# Autodesk Inventor assembly: Intake
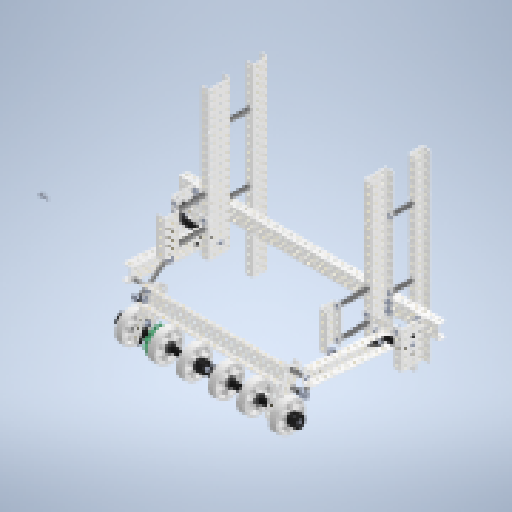
[picture p0: Inventor's stored thumbnail of the model, 512x512]
Saved by Autodesk Inventor 2023 (Build 270158000, 158)
## iProperties
Created: 2022-09-02
Part Number: Intake
Document SubType Name: Assembly
Designer: alex
Author: alex
## Documents named in this file (28)
- C:\Users\alex\Documents\GitHub\4067X_spin_up_cad\Mechanism\Intake.iam
- C:\Users\alex\Documents\GitHub\4067X_spin_up_cad\Library\Structure\Standoff\Standoff 1.00.ipt
- C:\Users\alex\Documents\GitHub\4067X_spin_up_cad\Library\Structure\Standoff.ipt
- C:\Users\alex\Documents\GitHub\4067X_spin_up_cad\Library\Structure\Standoff\Standoff 2.00.ipt
- C:\Users\alex\Documents\GitHub\4067X_spin_up_cad\Library\Structure\Hardware\Screw Steel - Star\SScrew Star Smooth .290.ipt
- C:\Users\alex\Documents\GitHub\4067X_spin_up_cad\Library\Structure\Hardware\Screw Steel - Star.ipt
- C:\Users\alex\Documents\GitHub\4067X_spin_up_cad\Library\Structure\Standoff\Standoff .50.ipt
- C:\Users\alex\Documents\GitHub\4067X_spin_up_cad\Library\Motion\Spacers\Spacer Nylon .375 OD.ipt
- C:\Users\alex\Documents\GitHub\4067X_spin_up_cad\Library\Structure\Hardware\Nut Keps.ipt
- C:\Users\alex\Documents\GitHub\4067X_spin_up_cad\Library\Motion\1-Post Bearing Flat Hex Retainer.ipt
- C:\Users\alex\Documents\GitHub\4067X_spin_up_cad\Library\Structure\Hardware\Screw Steel - Star\SScrew Star Smooth .375.ipt
- C:\Users\alex\Documents\GitHub\4067X_spin_up_cad\Library\Structure\Hardware\Nut Nylock.ipt
- C:\Users\alex\Documents\GitHub\4067X_spin_up_cad\Library\Structure\C-Channels\Aluminum 1x3x1\Alu C 1x3x1x20.ipt
- C:\Users\alex\Documents\GitHub\4067X_spin_up_cad\Library\Structure\C-Channels\Aluminum 1x3x1\Alu C 1x3x1x5.ipt
- C:\Users\alex\Documents\GitHub\4067X_spin_up_cad\Library\Structure\C-Channels\Aluminum 1x2x1\Alu C 1x2x1x35.ipt
- C:\Users\alex\Documents\GitHub\4067X_spin_up_cad\Library\Structure\Plates\Aluminum\VEX Plates\Alu Plate VEX 1x5.ipt
- C:\Users\alex\Documents\GitHub\4067X_spin_up_cad\Library\Structure\Hardware\Screw Steel - Star\SScrew Star Smooth 2.500.ipt
- C:\Users\alex\Documents\GitHub\4067X_spin_up_cad\Library\Motion\Spacers\Spacer Nylon .375 OD\NSpacer .375 OD x .375.ipt
- C:\Users\alex\Documents\GitHub\4067X_spin_up_cad\Library\Motion\Spacers\Washer Steel\SWasher .375 OD x .015625.ipt
- C:\Users\alex\Documents\GitHub\4067X_spin_up_cad\Library\Motion\Spacers\Washer Steel.ipt
- C:\Users\alex\Documents\GitHub\4067X_spin_up_cad\Library\Motion\Spacers\Spacer Nylon .375 OD\NSpacer .375 OD x .500.ipt
- C:\Users\alex\Documents\GitHub\4067X_spin_up_cad\Library\Structure\C-Channels\Aluminum 1x2x1\Alu C 1x2x1x25.ipt
- C:\Users\alex\Documents\GitHub\4067X_spin_up_cad\Library\Motion\Shaft HS\HS Bearing Flat.ipt
- C:\Users\alex\Documents\GitHub\4067X_spin_up_cad\Library\Structure\Hardware\Screw Steel - Star\SScrew Star Smooth .500.ipt
- C:\Users\alex\Documents\GitHub\4067X_spin_up_cad\Library\Structure\Hardware\Nut Thin Nylock.ipt
- C:\Users\alex\Documents\GitHub\4067X_spin_up_cad\Library\Structure\Hardware\Screw Steel - Star\SScrew Star Smooth .750.ipt
- C:\Users\alex\Documents\GitHub\4067X_spin_up_cad\Library\Structure\C-Channels\Aluminum 1x2x1\Alu C 1x2x1x5.ipt
- C:\Users\alex\Documents\GitHub\4067X_spin_up_cad\Mechanism\FloatingIntake.iam
## Components (84 placed, 23 different names)
1. Alu C 1x3x1x20:1 — Insert:105, Insert:106, Insert:109, Insert:113, Insert:115, Insert:116, Insert:117, Insert:231, Insert:234, Insert:235, Insert:238, Insert:241
2. Alu C 1x3x1x5:1 — Insert:107, Insert:108, Insert:114, Insert:120, Mate:15, Insert:145, Insert:230, Insert:244, Insert:245
3. Alu C 1x2x1x35:1 — Insert:105, Insert:106, Insert:107, Insert:108, Insert:126, Insert:127, Insert:150, Insert:151, Insert:218, Insert:219, Insert:222, Insert:223, Insert:232, Insert:233, Insert:236, Insert:237
4. Standoff 1.00:16 — Insert:109, Insert:110
5. Standoff .50:17 — Insert:110, Insert:125
6. Standoff 1.00:18 — Insert:113
7. Standoff .50:19 — Insert:124
8. Alu Plate VEX 1x5:1 — Insert:114, Insert:115, Insert:228, Insert:229
9. SScrew Star Smooth 2.500:31 — Insert:116
10. Nut Keps:3 — Insert:117, Insert:118
11. NSpacer .375 OD x .375:3 — Insert:119
12. SWasher .375 OD x .015625:1 — Insert:118, Insert:119
13. 1-Post Bearing Flat Hex Retainer:2 — Insert:120, Mate:15, Insert:146
14. NSpacer .375 OD x .500:4 — Insert:122
15. NSpacer .375 OD x .500:5 — Insert:122, Insert:123
16. NSpacer .375 OD x .375:6 — Insert:123
17. Alu C 1x2x1x25:1 — Insert:124, Insert:125, Insert:239, Insert:240
18. Alu C 1x3x1x20:2 — Insert:126, Insert:127, Insert:129, Insert:131, Insert:134, Insert:137, Insert:153, Insert:216, Insert:224, Insert:225, Insert:226, Insert:242, Insert:256, Insert:257, Mate:35
19. Standoff 1.00:20 — Insert:129
20. Standoff .50:21 — Insert:133
21. Standoff 1.00:22 — Insert:131
22. Standoff .50:23 — Insert:132
23. Alu C 1x2x1x25:2 — Insert:132, Insert:133, Insert:227, Insert:243
24. SScrew Star Smooth 2.500:32 — Insert:134, Mate:34
25. Nut Keps:4 — Insert:137
26. NSpacer .375 OD x .375:7
27. SWasher .375 OD x .015625:2
28. NSpacer .375 OD x .500:8
29. NSpacer .375 OD x .500:9
30. NSpacer .375 OD x .375:10
31. SScrew Star Smooth .375:34 — Insert:145
32. Nut Nylock:3 — Insert:146
33. Alu C 1x3x1x5:2 — Insert:150, Insert:151, Insert:152, Insert:217, Insert:220, Insert:221
34. 1-Post Bearing Flat Hex Retainer:4
35. SScrew Star Smooth .375:35
36. Nut Nylock:4
37. Alu Plate VEX 1x5:2 — Insert:152, Insert:153, Insert:214, Insert:215
38. SScrew Star Smooth .290:50 — Insert:214
39. SScrew Star Smooth .290:51 — Insert:215
40. Nut Keps:11 — Insert:216
41. Nut Keps:12 — Insert:217
42. SScrew Star Smooth .290:52 — Insert:218
43. SScrew Star Smooth .290:53 — Insert:219
44. Nut Keps:13 — Insert:220
45. Nut Keps:14 — Insert:221
46. SScrew Star Smooth .290:54 — Insert:222
47. SScrew Star Smooth .290:55 — Insert:223
48. Nut Keps:15 — Insert:224
49. Nut Keps:16 — Insert:225
50. SScrew Star Smooth .290:56 — Insert:226
51. SScrew Star Smooth .750:57 — Insert:227
52. SScrew Star Smooth .290:58 — Insert:228
53. SScrew Star Smooth .290:59 — Insert:229
54. Nut Keps:17 — Insert:230
55. Nut Keps:18 — Insert:231
56. SScrew Star Smooth .290:60 — Insert:232
57. SScrew Star Smooth .290:61 — Insert:233
58. Nut Keps:19 — Insert:234
59. Nut Keps:20 — Insert:235
60. SScrew Star Smooth .290:62 — Insert:236
61. SScrew Star Smooth .290:63 — Insert:237
62. SScrew Star Smooth .290:64 — Insert:238
63. SScrew Star Smooth .750:65 — Insert:239
64. SScrew Star Smooth .750:66 — Insert:240
65. SScrew Star Smooth .290:67 — Insert:241
66. SScrew Star Smooth .290:68 — Insert:242
67. SScrew Star Smooth .750:69 — Insert:243
68. Nut Keps:21 — Insert:244
69. Nut Keps:22 — Insert:245
70. Standoff 2.00:27 — Insert:249
71. Standoff 2.00:28 — Insert:248
72. Alu C 1x2x1x5:1 — Insert:248, Insert:249, Insert:250, Insert:251
73. SScrew Star Smooth .290:70 — Insert:250
74. SScrew Star Smooth .290:71 — Insert:251
75. Standoff 2.00:29 — Insert:256
76. Standoff 2.00:30 — Insert:257
77. Alu C 1x2x1x5:2 — Insert:259, Mate:33
78. SScrew Star Smooth .290:72
79. SScrew Star Smooth .290:73
80. HS Bearing Flat:3 — Insert:259, Mate:33, Insert:260
81. Nut Thin Nylock:3
82. SScrew Star Smooth .500:74
83. Nut Thin Nylock:4 — Insert:260
84. FloatingIntake:1 [sub-assembly] — Mate:34, Mate:35
## Relationships (94: Insert 89, Mate 5)
- Insert:105: Alu C 1x3x1x20:1 ↔ Alu C 1x2x1x35:1
- Insert:106: Alu C 1x3x1x20:1 ↔ Alu C 1x2x1x35:1
- Insert:107: Alu C 1x3x1x5:1 ↔ Alu C 1x2x1x35:1
- Insert:108: Alu C 1x3x1x5:1 ↔ Alu C 1x2x1x35:1
- Insert:109: Alu C 1x3x1x20:1 ↔ Standoff 1.00:16
- Insert:110: Standoff 1.00:16 ↔ Standoff .50:17
- [Insert]: Standoff 1.00:18 ↔ Standoff .50:19
- Insert:113: Alu C 1x3x1x20:1 ↔ Standoff 1.00:18
- Insert:114: Alu C 1x3x1x5:1 ↔ Alu Plate VEX 1x5:1
- Insert:115: Alu C 1x3x1x20:1 ↔ Alu Plate VEX 1x5:1
- Insert:116: Alu C 1x3x1x20:1 ↔ SScrew Star Smooth 2.500:31
- Insert:117: Alu C 1x3x1x20:1 ↔ Nut Keps:3
- Insert:118: Nut Keps:3 ↔ SWasher .375 OD x .015625:1
- Insert:119: NSpacer .375 OD x .375:3 ↔ SWasher .375 OD x .015625:1
- Insert:120: Alu C 1x3x1x5:1 ↔ 1-Post Bearing Flat Hex Retainer:2
- Mate:15: Alu C 1x3x1x5:1 ↔ 1-Post Bearing Flat Hex Retainer:2
- Insert:122: NSpacer .375 OD x .500:4 ↔ NSpacer .375 OD x .500:5
- Insert:123: NSpacer .375 OD x .500:5 ↔ NSpacer .375 OD x .375:6
- Insert:124: Standoff .50:19 ↔ Alu C 1x2x1x25:1
- Insert:125: Standoff .50:17 ↔ Alu C 1x2x1x25:1
- Insert:126: Alu C 1x2x1x35:1 ↔ Alu C 1x3x1x20:2
- Insert:127: Alu C 1x2x1x35:1 ↔ Alu C 1x3x1x20:2
- [Insert]: Standoff 1.00:20 ↔ Standoff .50:21
- Insert:129: Alu C 1x3x1x20:2 ↔ Standoff 1.00:20
- [Insert]: Standoff 1.00:22 ↔ Standoff .50:23
- Insert:131: Alu C 1x3x1x20:2 ↔ Standoff 1.00:22
- Insert:132: Standoff .50:23 ↔ Alu C 1x2x1x25:2
- Insert:133: Standoff .50:21 ↔ Alu C 1x2x1x25:2
- Insert:134: Alu C 1x3x1x20:2 ↔ SScrew Star Smooth 2.500:32
- [Insert]: Nut Keps:4 ↔ SWasher .375 OD x .015625:2
- [Insert]: NSpacer .375 OD x .375:7 ↔ SWasher .375 OD x .015625:2
- Insert:137: Alu C 1x3x1x20:2 ↔ Nut Keps:4
- [Insert]: NSpacer .375 OD x .500:8 ↔ NSpacer .375 OD x .500:9
- [Insert]: NSpacer .375 OD x .500:9 ↔ NSpacer .375 OD x .375:10
- Insert:145: Alu C 1x3x1x5:1 ↔ SScrew Star Smooth .375:34
- Insert:146: 1-Post Bearing Flat Hex Retainer:2 ↔ Nut Nylock:3
- [Insert]: Alu C 1x3x1x5:2 ↔ 1-Post Bearing Flat Hex Retainer:4
- [Mate]: Alu C 1x3x1x5:2 ↔ 1-Post Bearing Flat Hex Retainer:4
- [Insert]: Alu C 1x3x1x5:2 ↔ SScrew Star Smooth .375:35
- [Insert]: 1-Post Bearing Flat Hex Retainer:4 ↔ Nut Nylock:4
- Insert:150: Alu C 1x2x1x35:1 ↔ Alu C 1x3x1x5:2
- Insert:151: Alu C 1x2x1x35:1 ↔ Alu C 1x3x1x5:2
- Insert:152: Alu C 1x3x1x5:2 ↔ Alu Plate VEX 1x5:2
- Insert:153: Alu C 1x3x1x20:2 ↔ Alu Plate VEX 1x5:2
- Insert:214: Alu Plate VEX 1x5:2 ↔ SScrew Star Smooth .290:50
- Insert:215: Alu Plate VEX 1x5:2 ↔ SScrew Star Smooth .290:51
- Insert:216: Alu C 1x3x1x20:2 ↔ Nut Keps:11
- Insert:217: Alu C 1x3x1x5:2 ↔ Nut Keps:12
- Insert:218: Alu C 1x2x1x35:1 ↔ SScrew Star Smooth .290:52
- Insert:219: Alu C 1x2x1x35:1 ↔ SScrew Star Smooth .290:53
- Insert:220: Alu C 1x3x1x5:2 ↔ Nut Keps:13
- Insert:221: Alu C 1x3x1x5:2 ↔ Nut Keps:14
- Insert:222: Alu C 1x2x1x35:1 ↔ SScrew Star Smooth .290:54
- Insert:223: Alu C 1x2x1x35:1 ↔ SScrew Star Smooth .290:55
- Insert:224: Alu C 1x3x1x20:2 ↔ Nut Keps:15
- Insert:225: Alu C 1x3x1x20:2 ↔ Nut Keps:16
- Insert:226: Alu C 1x3x1x20:2 ↔ SScrew Star Smooth .290:56
- Insert:227: Alu C 1x2x1x25:2 ↔ SScrew Star Smooth .750:57
- Insert:228: Alu Plate VEX 1x5:1 ↔ SScrew Star Smooth .290:58
- Insert:229: Alu Plate VEX 1x5:1 ↔ SScrew Star Smooth .290:59
- Insert:230: Alu C 1x3x1x5:1 ↔ Nut Keps:17
- Insert:231: Alu C 1x3x1x20:1 ↔ Nut Keps:18
- Insert:232: Alu C 1x2x1x35:1 ↔ SScrew Star Smooth .290:60
- Insert:233: Alu C 1x2x1x35:1 ↔ SScrew Star Smooth .290:61
- Insert:234: Alu C 1x3x1x20:1 ↔ Nut Keps:19
- Insert:235: Alu C 1x3x1x20:1 ↔ Nut Keps:20
- Insert:236: Alu C 1x2x1x35:1 ↔ SScrew Star Smooth .290:62
- Insert:237: Alu C 1x2x1x35:1 ↔ SScrew Star Smooth .290:63
- Insert:238: Alu C 1x3x1x20:1 ↔ SScrew Star Smooth .290:64
- Insert:239: Alu C 1x2x1x25:1 ↔ SScrew Star Smooth .750:65
- Insert:240: Alu C 1x2x1x25:1 ↔ SScrew Star Smooth .750:66
- Insert:241: Alu C 1x3x1x20:1 ↔ SScrew Star Smooth .290:67
- Insert:242: Alu C 1x3x1x20:2 ↔ SScrew Star Smooth .290:68
- Insert:243: Alu C 1x2x1x25:2 ↔ SScrew Star Smooth .750:69
- Insert:244: Alu C 1x3x1x5:1 ↔ Nut Keps:21
- Insert:245: Alu C 1x3x1x5:1 ↔ Nut Keps:22
- [Insert]: Alu C 1x3x1x20:1 ↔ Standoff 2.00:27
- [Insert]: Alu C 1x3x1x20:1 ↔ Standoff 2.00:28
- Insert:248: Standoff 2.00:28 ↔ Alu C 1x2x1x5:1
- Insert:249: Standoff 2.00:27 ↔ Alu C 1x2x1x5:1
- Insert:250: Alu C 1x2x1x5:1 ↔ SScrew Star Smooth .290:70
- Insert:251: Alu C 1x2x1x5:1 ↔ SScrew Star Smooth .290:71
- [Insert]: Standoff 2.00:30 ↔ Alu C 1x2x1x5:2
- [Insert]: Standoff 2.00:29 ↔ Alu C 1x2x1x5:2
- [Insert]: Alu C 1x2x1x5:2 ↔ SScrew Star Smooth .290:72
- [Insert]: Alu C 1x2x1x5:2 ↔ SScrew Star Smooth .290:73
- Insert:256: Alu C 1x3x1x20:2 ↔ Standoff 2.00:29
- Insert:257: Alu C 1x3x1x20:2 ↔ Standoff 2.00:30
- [Insert]: HS Bearing Flat:3 ↔ Nut Thin Nylock:3
- Insert:259: Alu C 1x2x1x5:2 ↔ HS Bearing Flat:3
- Mate:33: Alu C 1x2x1x5:2 ↔ HS Bearing Flat:3
- Insert:260: HS Bearing Flat:3 ↔ Nut Thin Nylock:4
- Mate:34: SScrew Star Smooth 2.500:32 ↔ FloatingIntake:1
- Mate:35 (13.6398 mm): Alu C 1x3x1x20:2 ↔ FloatingIntake:1
## Named parameters: d171_d169 = 0 mm, d195_d169 = 0 mm, d197_d195_d169 = 0 mm, d202_d181 = 0 mm, d203_d182 = 0 mm, d210_d188 = 0 mm, d211_d189 = 0 mm, d215_d185 = 0 mm, d216_d186 = 0 mm, d217_d213 = 0 mm, d218_d214 = 0 mm, d351_d348 = 0 mm, d352_d349 = 0 mm, d353_d350 = 0 mm, d354_d347 = 0 mm, d357_d253_d244 = 0 mm
